# Autodesk Inventor assembly: arm
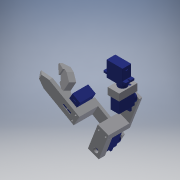
[picture p0: Inventor's stored thumbnail of the model, 180x180]
Saved by Autodesk Inventor 2018.3 (Build 223284000, 284)
## iProperties
Created: 2019-11-01
Part Number: arm
Material: 一般
Document SubType Name: Assembly
Designer: Eiji Nishizawa
Author: Eiji Nishizawa
## Documents named in this file (8)
- G:\OneDrive\CAD\arm\arm.iam
- G:\OneDrive\CAD\arm\armpart1.ipt
- G:\OneDrive\CAD\arm\armpart2.ipt
- G:\OneDrive\CAD\SG90\SG90 n.iam
- G:\OneDrive\CAD\arm\armpart3.ipt
- G:\OneDrive\CAD\arm\armpart4.ipt
- G:\OneDrive\CAD\arm\armmodulepart1.ipt
- G:\OneDrive\CAD\arm\armmodulepart2.ipt
## Components (10 placed, 7 different names)
1. armpart1:1 — 挿入:1, 挿入:2, 挿入:3, 挿入:4
2. armpart2:1 — 挿入:1, 挿入:2, 挿入:3, メイト:1, メイト:2, メイト:3
3. SG90 n:1 [sub-assembly] — メイト:1, メイト:2, メイト:3, 挿入:6
4. SG90 n:2 [sub-assembly] — 挿入:4, メイト:4, メイト:5, メイト:6
5. armpart3:1 — メイト:4, メイト:5, メイト:6, 挿入:5
6. SG90 n:3 [sub-assembly] — 挿入:5
7. armpart4:1 — 挿入:6, 挿入:7, 挿入:8, メイト:7
8. armmodulepart1:2 — 挿入:7, 挿入:8, メイト:8, メイト:9
9. SG90 n:4 [sub-assembly] — メイト:7, メイト:8, メイト:9, 挿入:9
10. armmodulepart2:1 — 挿入:9
## Relationships (18: Insert 9, Mate 9)
- 挿入:1 [Insert]: armpart1:1 ↔ armpart2:1
- 挿入:2 [Insert]: armpart1:1 ↔ armpart2:1
- 挿入:3 [Insert]: armpart1:1 ↔ armpart2:1
- メイト:1 [Mate]: armpart2:1 ↔ SG90 n:1
- メイト:2 [Mate]: armpart2:1 ↔ SG90 n:1
- 挿入:4 [Insert]: armpart1:1 ↔ SG90 n:2
- メイト:3 [Mate]: armpart2:1 ↔ SG90 n:1
- メイト:4 [Mate]: SG90 n:2 ↔ armpart3:1
- メイト:5 [Mate]: SG90 n:2 ↔ armpart3:1
- メイト:6 [Mate]: SG90 n:2 ↔ armpart3:1
- 挿入:5 [Insert]: armpart3:1 ↔ SG90 n:3
- 挿入:6 [Insert]: SG90 n:1 ↔ armpart4:1
- 挿入:7 [Insert]: armpart4:1 ↔ armmodulepart1:2
- 挿入:8 [Insert]: armpart4:1 ↔ armmodulepart1:2
- メイト:7 [Mate]: armpart4:1 ↔ SG90 n:4
- メイト:8 [Mate]: armmodulepart1:2 ↔ SG90 n:4
- メイト:9 [Mate]: armmodulepart1:2 ↔ SG90 n:4
- 挿入:9 [Insert]: SG90 n:4 ↔ armmodulepart2:1
